# Autodesk Inventor assembly: Electric-Scooter
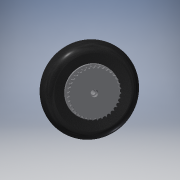
[picture p0: Inventor's stored thumbnail of the model, 180x180]
Saved by Autodesk Inventor 2018 (Build 220112000, 112)
## iProperties
Created: 2018-08-05
Part Number: Electric-Scooter
Document SubType Name: Assembly
Designer: ruben
Author: ruben
## Documents named in this file (3)
- C:\Users\ruben\Documents\Inventor\Electric-Scooter\Transmission\Transmission.iam
- C:\Users\ruben\Documents\Inventor\Electric-Scooter\Transmission\Sprocket 3-8x7-32 36T.ipt
- C:\Users\ruben\Documents\Inventor\Electric-Scooter\Wheels\Wheel.iam
## Components (2 placed, 2 different names)
1. Sprocket 3-8x7-32 36T:1 — Insert:1
2. Wheel:1 [sub-assembly] — Insert:1
## Relationships (1: Insert 1)
- Insert:1 (-20 mm): Sprocket 3-8x7-32 36T:1 ↔ Wheel:1
